# Autodesk Inventor assembly: Main_Assembly
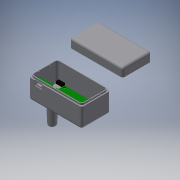
[picture p0: Inventor's stored thumbnail of the model, 180x180]
Saved by Autodesk Inventor 2017 (Build 210142000, 142)
## iProperties
Created: 2017-07-30
Part Number: Main_Assembly
Document SubType Name: Assembly
Designer: Mitch
Author: Mitch
## Documents named in this file (8)
- E:\Youtube Channel\Pojects\Brew Probe\Main_Assembly.iam
- E:\Youtube Channel\Pojects\Brew Probe\Bottom_Case.ipt
- E:\Youtube Channel\Pojects\Brew Probe\firebeetle_board.ipt
- E:\Youtube Channel\Pojects\Brew Probe\temp_probe_board.ipt
- E:\Youtube Channel\Pojects\Brew Probe\Top_Case.ipt
- E:\Youtube Channel\Pojects\Brew Probe\Insert.ipt
- E:\Youtube Channel\Pojects\Brew Probe\USB_Board_asy.iam
- E:\Youtube Channel\Pojects\Brew Probe\switch.ipt
## Components (7 placed, 7 different names)
1. Bottom_Case:1 — Mate:1, Mate:2, Mate:3, Mate:5, Mate:6, Mate:7, Mate:8, Flush:3, Mate:9, Mate:10
2. firebeetle_board:1 — Mate:1, Mate:2, Mate:3, Mate:4, Flush:1, Flush:2
3. temp_probe_board:1 — Mate:4, Flush:1, Flush:2
4. Top_Case:1
5. insert:1 — Mate:5, Mate:6
6. USB_Board_asy:1 [sub-assembly] — Mate:7, Mate:8, Mate:10
7. switch:1 — Flush:3, Mate:9
## Relationships (13: Mate 10, Flush 3)
- Mate:1 (1.27 mm): Bottom_Case:1 ↔ firebeetle_board:1
- Mate:2 (5.588 mm): Bottom_Case:1 ↔ firebeetle_board:1
- Mate:3 (1.27 mm): Bottom_Case:1 ↔ firebeetle_board:1
- Mate:4: firebeetle_board:1 ↔ temp_probe_board:1
- Flush:1 (6.985 mm): firebeetle_board:1 ↔ temp_probe_board:1
- Flush:2: firebeetle_board:1 ↔ temp_probe_board:1
- Mate:5: Bottom_Case:1 ↔ insert:1
- Mate:6: Bottom_Case:1 ↔ insert:1
- Mate:7: Bottom_Case:1 ↔ USB_Board_asy:1
- Mate:8 (1.27 mm): Bottom_Case:1 ↔ USB_Board_asy:1
- Flush:3: Bottom_Case:1 ↔ switch:1
- Mate:9 (1.27 mm): Bottom_Case:1 ↔ switch:1
- Mate:10: Bottom_Case:1 ↔ USB_Board_asy:1
